# Autodesk Inventor assembly: derive_casing_v2
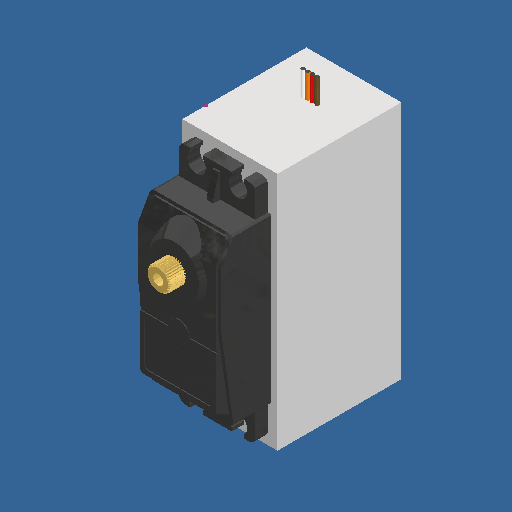
[picture p0: Inventor's stored thumbnail of the model, 512x512]
Saved by Autodesk Inventor 2026.2 (Build 302298000, 298)
## iProperties
Created: 2026-01-15
Part Number: derive_casing_v2
Document SubType Name: Assembly
Designer: Thoma
Author: Thoma
## Documents named in this file (3)
- C:\Users\Thoma\OneDrive\Desktop\dir\telescope_cover\cover\derive_casing_v2.iam
- C:\Users\Thoma\OneDrive\Desktop\dir\telescope_cover\cover\casing.ipt
- C:\Users\Thoma\OneDrive\Desktop\dir\telescope_cover\servo\DSS-M15S Servo.ipt
## Components (2 placed, 2 different names)
1. casing:1 — Mate:1, Flush:1, Flush:2
2. DSS-M15S Servo:1 — Mate:1, Flush:1, Flush:2
## Relationships (3: Flush 2, Mate 1)
- Mate:1: casing:1 ↔ DSS-M15S Servo:1
- Flush:1 (1.5 mm): casing:1 ↔ DSS-M15S Servo:1
- Flush:2 (2 mm): casing:1 ↔ DSS-M15S Servo:1
